# Autodesk Inventor assembly: Assembly Final
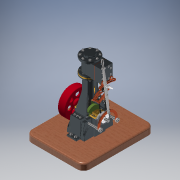
[picture p0: Inventor's stored thumbnail of the model, 180x180]
Saved by Autodesk Inventor 2017 (Build 210142000, 142)
## iProperties
Created: 2018-11-19
Part Number: Assembly Final
Document SubType Name: Assembly
Designer: Arman Grewal
Author: Arman Grewal
## Documents named in this file (56)
- C:\Users\Arman Grewal\Desktop\Engine\Assembly Final.iam
- C:\Users\Arman Grewal\Desktop\Engine\Piston.ipt
- C:\Users\Arman Grewal\Desktop\Engine\Piston Rod.ipt
- C:\Users\Arman Grewal\Documents\Inventor\Content Center Files\R2017\en-US\DIN 934\DIN 934 - M4 x 0.7.ipt
- C:\Users\Arman Grewal\Desktop\Engine\Crosshead.ipt
- C:\Users\Arman Grewal\Desktop\Engine\Crankrod.ipt
- C:\Users\Arman Grewal\Desktop\Engine\Crankrod Pin.ipt
- C:\Users\Arman Grewal\Desktop\Engine\Crankshaft outer rod.ipt
- C:\Users\Arman Grewal\Desktop\Engine\Crankshaft Center Rod.ipt
- C:\Users\Arman Grewal\Desktop\Engine\Crankshaft Counterweight.ipt
- C:\Users\Arman Grewal\Desktop\Engine\Vertical Steam Engine with Reverse Gear (anno 1830) Connecting Rod.ipt
- C:\Users\Arman Grewal\Desktop\Engine\Bearing Keeper.ipt
- C:\Users\Arman Grewal\Documents\Inventor\Content Center Files\R2017\en-US\DIN 84\DIN 84 - M3 x 8.ipt
- C:\Users\Arman Grewal\Desktop\Engine\Stand.ipt
- C:\Users\Arman Grewal\Desktop\Engine\Base cast f.ipt
- C:\Users\Arman Grewal\Documents\Inventor\Content Center Files\R2017\en-US\DIN 912\DIN 912 - M4 x 0.7 x 20 x 18.25.ipt
- C:\Users\Arman Grewal\Documents\Inventor\Content Center Files\R2017\en-US\DIN 6797  J\DIN 6797 - J 5.3.ipt
- C:\Users\Arman Grewal\Documents\Inventor\Content Center Files\R2017\en-US\DIN 934\DIN 934 - M5 x 0.8.ipt
- C:\Users\Arman Grewal\Desktop\Engine\Lower Base Bearing Holder.ipt
- C:\Users\Arman Grewal\Desktop\Engine\Upper Base Bearing Holder.ipt
- C:\Users\Arman Grewal\Documents\Inventor\Content Center Files\R2017\en-US\DIN 84\DIN 84 - M3 x 18.ipt
- C:\Users\Arman Grewal\Documents\Inventor\Content Center Files\R2017\en-US\DIN 84\DIN 84 - M3 x 20.ipt
- C:\Users\Arman Grewal\Desktop\Engine\Standard.ipt
- C:\Users\Arman Grewal\Desktop\Engine\cylinder.ipt
- C:\Users\Arman Grewal\Desktop\Engine\Upper Cylinder Cover.ipt
- C:\Users\Arman Grewal\Documents\Inventor\Content Center Files\R2017\en-US\DIN 912\DIN 912 - M3 x 0.5 x 16 x 14.75.ipt
- C:\Users\Arman Grewal\Documents\Inventor\Content Center Files\R2017\en-US\DIN 128\DIN 128 - A3.5.ipt
- C:\Users\Arman Grewal\Desktop\Engine\Lower Cylinder Cover.ipt
- C:\Users\Arman Grewal\Desktop\Engine\Upper Cylinder Packing.ipt
- C:\Users\Arman Grewal\Documents\Inventor\Content Center Files\R2017\en-US\DIN 912\DIN 912 - M3 x 0.5 x 12 x 10.75.ipt
- C:\Users\Arman Grewal\Desktop\Engine\Valve Plate.ipt
- C:\Users\Arman Grewal\Desktop\Engine\Steam Chest.ipt
- C:\Users\Arman Grewal\Desktop\Engine\Glands.ipt
- C:\Users\Arman Grewal\Desktop\Engine\Steam Chest Slide Valve Rod.ipt
- C:\Users\Arman Grewal\Desktop\Engine\Steam Chest Slide Valve.ipt
- C:\Users\Arman Grewal\Desktop\Engine\Steam Chest Cover.ipt
- C:\Users\Arman Grewal\Documents\Inventor\Content Center Files\R2017\en-US\DIN 84\DIN 84 - M2.5 x 10.ipt
- C:\Users\Arman Grewal\Documents\Inventor\Content Center Files\R2017\en-US\DIN 912\DIN 912 - M3 x 0.5 x 5 x 3.75.ipt
- C:\Users\Arman Grewal\Desktop\Engine\flywheel.ipt
- C:\Users\Arman Grewal\Desktop\Engine\Reverse Gear link 1.ipt
- C:\Users\Arman Grewal\Documents\Inventor\Content Center Files\R2017\en-US\DIN 7991(2)\DIN 7991 - M3x12.ipt
- C:\Users\Arman Grewal\Desktop\Engine\Reverse Lever.ipt
- C:\Users\Arman Grewal\Desktop\Engine\Reverse Gear Link Block.ipt
- C:\Users\Arman Grewal\Desktop\Engine\Reverse Gear Drag Link.ipt
- C:\Users\Arman Grewal\Desktop\Engine\Reverse Lever Ring Stud.ipt
- C:\Users\Arman Grewal\Desktop\Engine\Reverse Lever Ring.ipt
- C:\Users\Arman Grewal\Desktop\Engine\Reverse Gear Link Lever.ipt
- C:\Users\Arman Grewal\Desktop\Engine\Reverse Gear Link 1 updated.ipt
- C:\Users\Arman Grewal\Desktop\Engine\Reverse Gear LInk Rod.ipt
- C:\Users\Arman Grewal\Desktop\Engine\eccentric rod.ipt
- C:\Users\Arman Grewal\Desktop\Engine\eccentric.ipt
- C:\Users\Arman Grewal\Documents\Inventor\Content Center Files\R2017\en-US\DIN 84\DIN 84 - M2.5 x 8.ipt
- C:\Users\Arman Grewal\Desktop\Engine\Upper eccentric trap  lower eccentric trap (1).ipt
- C:\Users\Arman Grewal\Desktop\Engine\Upper lower eccentric trap (2).ipt
- C:\Users\Arman Grewal\Documents\Inventor\Content Center Files\R2017\en-US\AS 1427(01)\AS 1427 - M3 x 5(3).ipt
- C:\Users\Arman Grewal\Documents\Inventor\Content Center Files\R2017\en-US\DIN 934\DIN 934 - M6 x 1.ipt
## Components (140 placed, 55 different names)
1. Piston:1 — Mate:4, Insert:1, Angle:2, Mate:114, Mate:115
2. Piston Rod:1 — Mate:4, Mate:5, Mate:6, Mate:115, Mate:122
3. DIN 934 - replaced by DIN EN 24032/28673/28674 M4:1 — Insert:1
4. Crosshead:1 — Mate:5, Mate:6, Mate:7, Mate:8
5. Crankrod:1 — Mate:7, Mate:8, Mate:9, Mate:11, Mate:12
6. Crankrod Pin:1 — Mate:9
7. Crankshaft outer rod:1 — Mate:23, Mate:24, Mate:52, Mate:156, Mate:162, Rotation:2, Rotation:3
8. Crankshaft outer rod:2 — Mate:21, Mate:22, Mate:108, Flush:3
9. Crankshaft Center Rod:1 — Mate:20, Mate:25, Mate:26, Mate:27, Mate:28
10. Crankshaft Counterweight:1 — Mate:23, Mate:24, Mate:27, Mate:28, Mate:53, Rotation:1
11. Crankshaft Counterweight:2 — Mate:21, Mate:22, Mate:25, Mate:26, Mate:29
12. Vertical Steam Engine with Reverse Gear (anno 1830) Connecting Rod:1 — Mate:14, Mate:15, Mate:16, Mate:17, Mate:18, Mate:19, Mate:20, Mate:29
13. Vertical Steam Engine with Reverse Gear (anno 1830) Connecting Rod:2 — Mate:11, Mate:12, Mate:14, Mate:15, Mate:16
14. Bearing Keeper:1 — Mate:17, Mate:18, Mate:19, Insert:2, Insert:3
15. DIN 84 - replaced by DIN EN ISO 1207 M3 x 8:1 — Insert:2
16. DIN 84 - replaced by DIN EN ISO 1207 M3 x 8:2 — Insert:3
17. Stand:1 — Mate:30, Mate:31, Mate:32, Mate:33, Insert:8, Insert:9, Insert:10, Insert:11, Mate:34, Mate:36, Mate:38, Mate:40, Angle:1
18. Base cast f:1 — Mate:30, Mate:31, Mate:32, Mate:33, Insert:4, Insert:5, Insert:6, Insert:7, Mate:48, Flush:1, Mate:49, Mate:50, Flush:2, Mate:51, Mate:53, Mate:55, Mate:56, Mate:57, Mate:58, Mate:60, Mate:61, Mate:62, Mate:63, Mate:64, Mate:65, Mate:66, Mate:125, Mate:126, Mate:127, Mate:128
19. DIN 912 - replaced by DIN EN ISO 4762 M4 x 20:1 — Insert:4, Mate:42
20. DIN 912 - replaced by DIN EN ISO 4762 M4 x 20:2 — Insert:5, Mate:44
21. DIN 912 - replaced by DIN EN ISO 4762 M4 x 20:3 — Insert:6, Mate:46
22. DIN 912 - replaced by DIN EN ISO 4762 M4 x 20:4 — Insert:7
23. DIN 6797 J J 5.3:1 — Insert:8
24. DIN 6797 J J 5.3:2 — Insert:9
25. DIN 6797 J J 5.3:3 — Insert:10
26. DIN 6797 J J 5.3:4 — Insert:11, Mate:35, Mate:37, Mate:39, Mate:41
27. DIN 6797 J J 5.3:5 — Mate:34, Mate:35, Mate:43
28. DIN 6797 J J 5.3:6 — Mate:36, Mate:37, Mate:47
29. DIN 6797 J J 5.3:7 — Mate:38, Mate:39, Mate:45
30. DIN 6797 J J 5.3:8 — Mate:40, Mate:41, Insert:12, Insert:13, Insert:14, Insert:15, Insert:16, Insert:17, Insert:18, Insert:19
31. DIN 934 - replaced by DIN EN 24032/28673/28674 M5:1 — Insert:12
32. DIN 934 - replaced by DIN EN 24032/28673/28674 M5:2 — Insert:13
33. DIN 934 - replaced by DIN EN 24032/28673/28674 M5:3 — Insert:14
34. DIN 934 - replaced by DIN EN 24032/28673/28674 M5:4 — Insert:15
35. DIN 934 - replaced by DIN EN 24032/28673/28674 M5:5 — Insert:16
36. DIN 934 - replaced by DIN EN 24032/28673/28674 M5:6 — Insert:17
37. DIN 934 - replaced by DIN EN 24032/28673/28674 M5:7 — Insert:18
38. DIN 934 - replaced by DIN EN 24032/28673/28674 M5:8 — Insert:19
39. DIN 934 - replaced by DIN EN 24032/28673/28674 M4:2 — Mate:42, Mate:43
40. DIN 934 - replaced by DIN EN 24032/28673/28674 M4:3 — Mate:44, Mate:45
41. DIN 934 - replaced by DIN EN 24032/28673/28674 M4:4 — Mate:46, Mate:47
42. Lower Base Bearing Holder:1 — Mate:50, Flush:2, Mate:51, Mate:52, Mate:54
43. Lower Base Bearing Holder:2 — Mate:48, Flush:1, Mate:49, Mate:59
44. Upper Base Bearing Holder:1 — Mate:59, Mate:60, Mate:61, Mate:62, Mate:63, Insert:24, Insert:25, Insert:26, Insert:27
45. Upper Base Bearing Holder:2 — Mate:54, Mate:55, Mate:56, Mate:57, Mate:58, Insert:28, Insert:29, Insert:30, Insert:31
46. DIN 84 - replaced by DIN EN ISO 1207 M3 x 18:1 — Insert:24
47. DIN 84 - replaced by DIN EN ISO 1207 M3 x 18:2 — Insert:25
48. DIN 84 - replaced by DIN EN ISO 1207 M3 x 18:3 — Insert:26
49. DIN 84 - replaced by DIN EN ISO 1207 M3 x 18:4 — Insert:27
50. DIN 84 - replaced by DIN EN ISO 1207 M3 x 20:1 — Insert:28
51. DIN 84 - replaced by DIN EN ISO 1207 M3 x 20:2 — Insert:29
52. DIN 84 - replaced by DIN EN ISO 1207 M3 x 20:3 — Insert:30
53. DIN 84 - replaced by DIN EN ISO 1207 M3 x 20:4 — Insert:31
54. Standard:1 — Mate:64, Mate:65, Mate:66, Insert:32, Insert:33, Insert:34, Insert:35, Insert:36, Insert:37, Insert:38, Insert:39, Insert:40, Insert:41, Insert:42, Insert:43, Insert:44, Insert:45, Mate:67, Mate:68, Mate:69, Mate:70, Mate:71
55. DIN 912 - replaced by DIN EN ISO 4762 M3 x 16:1 — Insert:32
56. DIN 912 - replaced by DIN EN ISO 4762 M3 x 16:2 — Insert:33
57. DIN 912 - replaced by DIN EN ISO 4762 M3 x 16:3 — Insert:34
58. DIN 912 - replaced by DIN EN ISO 4762 M3 x 16:4 — Insert:35
59. DIN 912 - replaced by DIN EN ISO 4762 M3 x 16:5 — Insert:36
60. DIN 912 - replaced by DIN EN ISO 4762 M3 x 16:6 — Insert:37
61. DIN 128 A3.5:1 — Insert:38, Insert:50
62. DIN 128 A3.5:2 — Insert:39, Insert:49
63. DIN 128 A3.5:3 — Insert:40, Insert:51
64. DIN 128 A3.5:4 — Insert:41, Insert:46
65. DIN 128 A3.5:5 — Insert:42, Insert:47
66. DIN 128 A3.5:6 — Insert:43, Insert:52
67. DIN 128 A3.5:7 — Insert:44, Mate:85, Mate:86
68. DIN 128 A3.5:8 — Insert:45, Insert:48
69. Lower Cylinder Cover:1 — Mate:67, Mate:68, Mate:69, Mate:70, Mate:71, Mate:72, Mate:73, Mate:74, Mate:75, Mate:76, Mate:77, Mate:122
70. cylinder:1 — Mate:72, Angle:1, Mate:73, Mate:74, Mate:75, Mate:76, Mate:77, Angle:2, Mate:78, Mate:79, Mate:80, Mate:82, Mate:83, Mate:84, Mate:87, Mate:88, Mate:89, Mate:91, Mate:92, Mate:114
71. Upper Cylinder Packing:1 — Mate:78, Mate:79, Mate:80, Mate:81
72. Upper Cylinder Cover:1 — Mate:81, Mate:82, Mate:83, Mate:84, Insert:53, Insert:54, Insert:55, Insert:56, Insert:57, Insert:58, Insert:59, Insert:60, Insert:66
73. DIN 912 - replaced by DIN EN ISO 4762 M3 x 12:1 — Insert:46
74. DIN 912 - replaced by DIN EN ISO 4762 M3 x 12:2 — Mate:85, Mate:86
75. DIN 912 - replaced by DIN EN ISO 4762 M3 x 12:3 — Insert:47
76. DIN 912 - replaced by DIN EN ISO 4762 M3 x 12:4 — Insert:48
77. DIN 912 - replaced by DIN EN ISO 4762 M3 x 12:5 — Insert:49
78. DIN 912 - replaced by DIN EN ISO 4762 M3 x 12:6 — Insert:50
79. DIN 912 - replaced by DIN EN ISO 4762 M3 x 12:7 — Insert:51
80. DIN 912 - replaced by DIN EN ISO 4762 M3 x 12:8 — Insert:52
81. Valve Plate:1 — Mate:87, Mate:88, Mate:89, Mate:90, Mate:98
82. Steam Chest:1 — Mate:90, Mate:91, Mate:92, Mate:93, Mate:94, Mate:95, Angle:3, Angle:4, Mate:104, Mate:105, Mate:107, Mate:116
83. Glands:1 — Mate:93, Mate:94, Mate:95, Mate:99, Insert:69, Insert:70
84. DIN 128 A3.5:9 — Insert:53, Insert:61
85. DIN 128 A3.5:10 — Insert:54, Insert:63
86. DIN 128 A3.5:11 — Insert:55, Insert:62
87. DIN 128 A3.5:12 — Insert:56, Insert:64
88. DIN 128 A3.5:13 — Insert:57, Insert:68
89. DIN 128 A3.5:14 — Insert:58
90. DIN 128 A3.5:15 — Insert:59, Insert:67
91. DIN 128 A3.5:16 — Insert:60, Insert:65
92. DIN 912 - replaced by DIN EN ISO 4762 M3 x 12:9 — Insert:61
93. DIN 912 - replaced by DIN EN ISO 4762 M3 x 12:10 — Insert:62
94. DIN 912 - replaced by DIN EN ISO 4762 M3 x 12:11 — Insert:63
95. DIN 912 - replaced by DIN EN ISO 4762 M3 x 12:12 — Insert:64
96. DIN 912 - replaced by DIN EN ISO 4762 M3 x 12:13 — Insert:65
97. DIN 912 - replaced by DIN EN ISO 4762 M3 x 12:14 — Insert:66
98. DIN 912 - replaced by DIN EN ISO 4762 M3 x 12:15 — Insert:67
99. DIN 912 - replaced by DIN EN ISO 4762 M3 x 12:16 — Insert:68
100. Steam Chest Slide Valve Rod:1 — Mate:96, Mate:97, Angle:4, Mate:99, Mate:100, Mate:102, Mate:139, Mate:140
101. Steam Chest Slide Valve:1 — Mate:96, Mate:97, Mate:98, Angle:3, Mate:101, Mate:103, Mate:116
102. DIN 934 - replaced by DIN EN 24032/28673/28674 M4:5 — Mate:100, Mate:101
103. DIN 934 - replaced by DIN EN 24032/28673/28674 M4:6 — Mate:102, Mate:103
104. Steam Chest Cover:1 — Mate:104, Mate:105, Mate:107, Insert:71, Insert:72, Insert:73, Insert:74, Insert:75, Insert:76, Insert:77, Insert:78, Mate:117, Mate:118, Mate:119
105. DIN 84 - replaced by DIN EN ISO 1207 M2.5 x 10:1 — Insert:69
106. DIN 84 - replaced by DIN EN ISO 1207 M2.5 x 10:2 — Insert:70
107. DIN 912 - replaced by DIN EN ISO 4762 M3 x 5:1 — Insert:71
108. DIN 912 - replaced by DIN EN ISO 4762 M3 x 5:2 — Insert:72
109. DIN 912 - replaced by DIN EN ISO 4762 M3 x 5:3 — Insert:73
110. DIN 912 - replaced by DIN EN ISO 4762 M3 x 5:4 — Insert:74
111. DIN 912 - replaced by DIN EN ISO 4762 M3 x 5:5 — Insert:75
112. DIN 912 - replaced by DIN EN ISO 4762 M3 x 5:6 — Insert:76
113. DIN 912 - replaced by DIN EN ISO 4762 M3 x 5:7 — Insert:77
114. DIN 912 - replaced by DIN EN ISO 4762 M3 x 5:8 — Insert:78
115. flywheel:1 — Mate:108, Flush:3, Rotation:1
116. Reverse Lever:1 — Mate:123, Mate:124, Mate:132, Mate:133, Mate:134, Mate:146, Insert:81
117. Reverse Gear link 1:1 — Mate:117, Mate:118, Mate:119, Mate:120, Mate:121
118. DIN 7991 M3x12:1 — Mate:120
119. DIN 7991 M3x12:2 — Mate:121
120. Reverse Gear Drag Link:1 — Mate:123, Mate:124, Mate:163, Mate:164, Mate:165
121. Reverse Lever Ring Stud:1 — Mate:127, Mate:128, Mate:130, Mate:168
122. Reverse Lever Ring Stud:2 — Mate:125, Mate:126, Mate:129, Mate:166
123. Reverse Lever Ring:1 — Mate:129, Mate:130, Mate:132, Mate:146, Mate:167, Mate:169
124. Reverse Gear Link Lever:1 — Mate:133, Mate:134
125. Reverse Gear Link 1 updated:1 — Mate:138, Flush:4, Mate:141, Mate:143, Mate:147, Mate:148, Mate:149, Mate:150
126. Reverse Gear Link Block:1 — Mate:138, Flush:4, Mate:139, Mate:140
127. Reverse Gear LInk Rod:1 — Mate:141, Mate:143, Mate:163, Mate:164, Mate:165
128. eccentric rod:1 — Mate:147, Mate:148, Insert:79, Mate:154, Mate:155
129. eccentric rod:2 — Mate:149, Mate:150, Insert:80, Mate:160, Mate:161
130. DIN 84 - replaced by DIN EN ISO 1207 M2.5 x 8:1 — Insert:79
131. DIN 84 - replaced by DIN EN ISO 1207 M2.5 x 8:2 — Insert:80
132. Upper lower eccentric trap (2):3 — Mate:152, Mate:153, Flush:5
133. Upper eccentric trap  lower eccentric trap (1):1 — Mate:151, Mate:153, Flush:6, Mate:154, Mate:155
134. eccentric:1 — Mate:151, Mate:152, Flush:5, Flush:6, Mate:156, Rotation:3
135. eccentric:2 — Mate:157, Mate:158, Flush:7, Flush:8, Mate:162, Rotation:2
136. Upper lower eccentric trap (2):4 — Mate:158, Mate:159, Flush:8
137. Upper eccentric trap  lower eccentric trap (1):2 — Mate:157, Mate:159, Flush:7, Mate:160, Mate:161
138. AS 1427 - Metric M3 x 5:1 — Insert:81
139. DIN 934 - replaced by DIN EN 24032/28673/28674 M6:1 — Mate:166, Mate:167
140. DIN 934 - replaced by DIN EN 24032/28673/28674 M6:2 — Mate:168, Mate:169
## Relationships (243: Mate 151, Insert 77, Flush 8, Angle 4, RelateRotation 3)
- Mate:4: Piston:1 ↔ Piston Rod:1
- Insert:1: Piston:1 ↔ DIN 934 - replaced by DIN EN 24032/28673/28674 M4:1
- Mate:5: Piston Rod:1 ↔ Crosshead:1
- Mate:6 (-7.628 mm): Piston Rod:1 ↔ Crosshead:1
- Mate:7: Crosshead:1 ↔ Crankrod:1
- Mate:8: Crosshead:1 ↔ Crankrod:1
- Mate:9: Crankrod:1 ↔ Crankrod Pin:1
- Mate:11: Crankrod:1 ↔ Vertical Steam Engine with Reverse Gear (anno 1830) Connecting Rod:2
- Mate:12: Crankrod:1 ↔ Vertical Steam Engine with Reverse Gear (anno 1830) Connecting Rod:2
- Mate:14: Vertical Steam Engine with Reverse Gear (anno 1830) Connecting Rod:1 ↔ Vertical Steam Engine with Reverse Gear (anno 1830) Connecting Rod:2
- Mate:15: Vertical Steam Engine with Reverse Gear (anno 1830) Connecting Rod:1 ↔ Vertical Steam Engine with Reverse Gear (anno 1830) Connecting Rod:2
- Mate:16: Vertical Steam Engine with Reverse Gear (anno 1830) Connecting Rod:1 ↔ Vertical Steam Engine with Reverse Gear (anno 1830) Connecting Rod:2
- Mate:17: Vertical Steam Engine with Reverse Gear (anno 1830) Connecting Rod:1 ↔ Bearing Keeper:1
- Mate:18: Vertical Steam Engine with Reverse Gear (anno 1830) Connecting Rod:1 ↔ Bearing Keeper:1
- Mate:19: Vertical Steam Engine with Reverse Gear (anno 1830) Connecting Rod:1 ↔ Bearing Keeper:1
- Mate:20: Crankshaft Center Rod:1 ↔ Vertical Steam Engine with Reverse Gear (anno 1830) Connecting Rod:1
- Mate:21: Crankshaft outer rod:2 ↔ Crankshaft Counterweight:2
- Mate:22: Crankshaft outer rod:2 ↔ Crankshaft Counterweight:2
- Mate:23: Crankshaft outer rod:1 ↔ Crankshaft Counterweight:1
- Mate:24: Crankshaft outer rod:1 ↔ Crankshaft Counterweight:1
- Mate:25: Crankshaft Center Rod:1 ↔ Crankshaft Counterweight:2
- Mate:26: Crankshaft Center Rod:1 ↔ Crankshaft Counterweight:2
- Mate:27: Crankshaft Center Rod:1 ↔ Crankshaft Counterweight:1
- Mate:28: Crankshaft Center Rod:1 ↔ Crankshaft Counterweight:1
- Mate:29 (0.5 mm): Crankshaft Counterweight:2 ↔ Vertical Steam Engine with Reverse Gear (anno 1830) Connecting Rod:1
- Insert:2: Bearing Keeper:1 ↔ DIN 84 - replaced by DIN EN ISO 1207 M3 x 8:1
- Insert:3: Bearing Keeper:1 ↔ DIN 84 - replaced by DIN EN ISO 1207 M3 x 8:2
- Mate:30: Stand:1 ↔ Base cast f:1
- Mate:31: Stand:1 ↔ Base cast f:1
- Mate:32: Stand:1 ↔ Base cast f:1
- Mate:33: Stand:1 ↔ Base cast f:1
- Insert:4: Base cast f:1 ↔ DIN 912 - replaced by DIN EN ISO 4762 M4 x 20:1
- Insert:5: Base cast f:1 ↔ DIN 912 - replaced by DIN EN ISO 4762 M4 x 20:2
- Insert:6: Base cast f:1 ↔ DIN 912 - replaced by DIN EN ISO 4762 M4 x 20:3
- Insert:7: Base cast f:1 ↔ DIN 912 - replaced by DIN EN ISO 4762 M4 x 20:4
- Insert:8: Stand:1 ↔ DIN 6797 J J 5.3:1
- Insert:9: Stand:1 ↔ DIN 6797 J J 5.3:2
- Insert:10: Stand:1 ↔ DIN 6797 J J 5.3:3
- Insert:11: Stand:1 ↔ DIN 6797 J J 5.3:4
- Mate:34: Stand:1 ↔ DIN 6797 J J 5.3:5
- Mate:35: DIN 6797 J J 5.3:4 ↔ DIN 6797 J J 5.3:5
- Mate:36: Stand:1 ↔ DIN 6797 J J 5.3:6
- Mate:37: DIN 6797 J J 5.3:4 ↔ DIN 6797 J J 5.3:6
- Mate:38: Stand:1 ↔ DIN 6797 J J 5.3:7
- Mate:39: DIN 6797 J J 5.3:4 ↔ DIN 6797 J J 5.3:7
- Mate:40: Stand:1 ↔ DIN 6797 J J 5.3:8
- Mate:41: DIN 6797 J J 5.3:4 ↔ DIN 6797 J J 5.3:8
- Insert:12: DIN 6797 J J 5.3:8 ↔ DIN 934 - replaced by DIN EN 24032/28673/28674 M5:1
- Insert:13: DIN 6797 J J 5.3:8 ↔ DIN 934 - replaced by DIN EN 24032/28673/28674 M5:2
- Insert:14: DIN 6797 J J 5.3:8 ↔ DIN 934 - replaced by DIN EN 24032/28673/28674 M5:3
- Insert:15: DIN 6797 J J 5.3:8 ↔ DIN 934 - replaced by DIN EN 24032/28673/28674 M5:4
- Insert:16: DIN 6797 J J 5.3:8 ↔ DIN 934 - replaced by DIN EN 24032/28673/28674 M5:5
- Insert:17: DIN 6797 J J 5.3:8 ↔ DIN 934 - replaced by DIN EN 24032/28673/28674 M5:6
- Insert:18: DIN 6797 J J 5.3:8 ↔ DIN 934 - replaced by DIN EN 24032/28673/28674 M5:7
- Insert:19: DIN 6797 J J 5.3:8 ↔ DIN 934 - replaced by DIN EN 24032/28673/28674 M5:8
- Mate:42: DIN 912 - replaced by DIN EN ISO 4762 M4 x 20:1 ↔ DIN 934 - replaced by DIN EN 24032/28673/28674 M4:2
- Mate:43: DIN 6797 J J 5.3:5 ↔ DIN 934 - replaced by DIN EN 24032/28673/28674 M4:2
- Mate:44: DIN 912 - replaced by DIN EN ISO 4762 M4 x 20:2 ↔ DIN 934 - replaced by DIN EN 24032/28673/28674 M4:3
- Mate:45: DIN 6797 J J 5.3:7 ↔ DIN 934 - replaced by DIN EN 24032/28673/28674 M4:3
- Mate:46: DIN 912 - replaced by DIN EN ISO 4762 M4 x 20:3 ↔ DIN 934 - replaced by DIN EN 24032/28673/28674 M4:4
- Mate:47: DIN 6797 J J 5.3:6 ↔ DIN 934 - replaced by DIN EN 24032/28673/28674 M4:4
- Mate:48: Base cast f:1 ↔ Lower Base Bearing Holder:2
- Flush:1: Base cast f:1 ↔ Lower Base Bearing Holder:2
- Mate:49: Base cast f:1 ↔ Lower Base Bearing Holder:2
- Mate:50: Base cast f:1 ↔ Lower Base Bearing Holder:1
- Flush:2: Base cast f:1 ↔ Lower Base Bearing Holder:1
- Mate:51: Base cast f:1 ↔ Lower Base Bearing Holder:1
- Mate:52: Crankshaft outer rod:1 ↔ Lower Base Bearing Holder:1
- Mate:53 (2.5 mm): Crankshaft Counterweight:1 ↔ Base cast f:1
- Mate:54: Lower Base Bearing Holder:1 ↔ Upper Base Bearing Holder:2
- Mate:55: Base cast f:1 ↔ Upper Base Bearing Holder:2
- Mate:56: Base cast f:1 ↔ Upper Base Bearing Holder:2
- Mate:57: Base cast f:1 ↔ Upper Base Bearing Holder:2
- Mate:58: Base cast f:1 ↔ Upper Base Bearing Holder:2
- Mate:59: Lower Base Bearing Holder:2 ↔ Upper Base Bearing Holder:1
- Mate:60: Base cast f:1 ↔ Upper Base Bearing Holder:1
- Mate:61: Base cast f:1 ↔ Upper Base Bearing Holder:1
- Mate:62: Base cast f:1 ↔ Upper Base Bearing Holder:1
- Mate:63: Base cast f:1 ↔ Upper Base Bearing Holder:1
- Insert:24: Upper Base Bearing Holder:1 ↔ DIN 84 - replaced by DIN EN ISO 1207 M3 x 18:1
- Insert:25: Upper Base Bearing Holder:1 ↔ DIN 84 - replaced by DIN EN ISO 1207 M3 x 18:2
- Insert:26: Upper Base Bearing Holder:1 ↔ DIN 84 - replaced by DIN EN ISO 1207 M3 x 18:3
- Insert:27: Upper Base Bearing Holder:1 ↔ DIN 84 - replaced by DIN EN ISO 1207 M3 x 18:4
- Insert:28: Upper Base Bearing Holder:2 ↔ DIN 84 - replaced by DIN EN ISO 1207 M3 x 20:1
- Insert:29: Upper Base Bearing Holder:2 ↔ DIN 84 - replaced by DIN EN ISO 1207 M3 x 20:2
- Insert:30: Upper Base Bearing Holder:2 ↔ DIN 84 - replaced by DIN EN ISO 1207 M3 x 20:3
- Insert:31: Upper Base Bearing Holder:2 ↔ DIN 84 - replaced by DIN EN ISO 1207 M3 x 20:4
- Mate:64: Base cast f:1 ↔ Standard:1
- Mate:65: Base cast f:1 ↔ Standard:1
- Mate:66: Base cast f:1 ↔ Standard:1
- Insert:32: Standard:1 ↔ DIN 912 - replaced by DIN EN ISO 4762 M3 x 16:1
- Insert:33: Standard:1 ↔ DIN 912 - replaced by DIN EN ISO 4762 M3 x 16:2
- Insert:34: Standard:1 ↔ DIN 912 - replaced by DIN EN ISO 4762 M3 x 16:3
- Insert:35: Standard:1 ↔ DIN 912 - replaced by DIN EN ISO 4762 M3 x 16:4
- Insert:36: Standard:1 ↔ DIN 912 - replaced by DIN EN ISO 4762 M3 x 16:5
- Insert:37: Standard:1 ↔ DIN 912 - replaced by DIN EN ISO 4762 M3 x 16:6
- Insert:38: Standard:1 ↔ DIN 128 A3.5:1
- Insert:39: Standard:1 ↔ DIN 128 A3.5:2
- Insert:40: Standard:1 ↔ DIN 128 A3.5:3
- Insert:41: Standard:1 ↔ DIN 128 A3.5:4
- Insert:42: Standard:1 ↔ DIN 128 A3.5:5
- Insert:43: Standard:1 ↔ DIN 128 A3.5:6
- Insert:44: Standard:1 ↔ DIN 128 A3.5:7
- Insert:45: Standard:1 ↔ DIN 128 A3.5:8
- Mate:67: Standard:1 ↔ Lower Cylinder Cover:1
- Mate:68: Standard:1 ↔ Lower Cylinder Cover:1
- Mate:69: Standard:1 ↔ Lower Cylinder Cover:1
- Mate:70: Standard:1 ↔ Lower Cylinder Cover:1
- Mate:71: Standard:1 ↔ Lower Cylinder Cover:1
- Mate:72: Lower Cylinder Cover:1 ↔ cylinder:1
- Angle:1 (0 deg): Stand:1 ↔ cylinder:1
- Mate:73: Lower Cylinder Cover:1 ↔ cylinder:1
- Mate:74: Lower Cylinder Cover:1 ↔ cylinder:1
- Mate:75: Lower Cylinder Cover:1 ↔ cylinder:1
- Mate:76: Lower Cylinder Cover:1 ↔ cylinder:1
- Mate:77: Lower Cylinder Cover:1 ↔ cylinder:1
- Angle:2 (0 deg): Piston:1 ↔ cylinder:1
- Mate:78: cylinder:1 ↔ Upper Cylinder Packing:1
- Mate:79: cylinder:1 ↔ Upper Cylinder Packing:1
- Mate:80: cylinder:1 ↔ Upper Cylinder Packing:1
- Mate:81: Upper Cylinder Packing:1 ↔ Upper Cylinder Cover:1
- Mate:82: cylinder:1 ↔ Upper Cylinder Cover:1
- Mate:83: cylinder:1 ↔ Upper Cylinder Cover:1
- Mate:84: cylinder:1 ↔ Upper Cylinder Cover:1
- Insert:46: DIN 128 A3.5:4 ↔ DIN 912 - replaced by DIN EN ISO 4762 M3 x 12:1
- Mate:85: DIN 128 A3.5:7 ↔ DIN 912 - replaced by DIN EN ISO 4762 M3 x 12:2
- Mate:86: DIN 128 A3.5:7 ↔ DIN 912 - replaced by DIN EN ISO 4762 M3 x 12:2
- Insert:47: DIN 128 A3.5:5 ↔ DIN 912 - replaced by DIN EN ISO 4762 M3 x 12:3
- Insert:48: DIN 128 A3.5:8 ↔ DIN 912 - replaced by DIN EN ISO 4762 M3 x 12:4
- Insert:49: DIN 128 A3.5:2 ↔ DIN 912 - replaced by DIN EN ISO 4762 M3 x 12:5
- Insert:50: DIN 128 A3.5:1 ↔ DIN 912 - replaced by DIN EN ISO 4762 M3 x 12:6
- Insert:51: DIN 128 A3.5:3 ↔ DIN 912 - replaced by DIN EN ISO 4762 M3 x 12:7
- Insert:52: DIN 128 A3.5:6 ↔ DIN 912 - replaced by DIN EN ISO 4762 M3 x 12:8
- Mate:87: cylinder:1 ↔ Valve Plate:1
- Mate:88: cylinder:1 ↔ Valve Plate:1
- Mate:89: cylinder:1 ↔ Valve Plate:1
- Mate:90: Valve Plate:1 ↔ Steam Chest:1
- Mate:91: cylinder:1 ↔ Steam Chest:1
- Mate:92: cylinder:1 ↔ Steam Chest:1
- Mate:93: Steam Chest:1 ↔ Glands:1
- Mate:94: Steam Chest:1 ↔ Glands:1
- Mate:95: Steam Chest:1 ↔ Glands:1
- Insert:53: Upper Cylinder Cover:1 ↔ DIN 128 A3.5:9
- Insert:54: Upper Cylinder Cover:1 ↔ DIN 128 A3.5:10
- Insert:55: Upper Cylinder Cover:1 ↔ DIN 128 A3.5:11
- Insert:56: Upper Cylinder Cover:1 ↔ DIN 128 A3.5:12
- Insert:57: Upper Cylinder Cover:1 ↔ DIN 128 A3.5:13
- Insert:58: Upper Cylinder Cover:1 ↔ DIN 128 A3.5:14
- Insert:59: Upper Cylinder Cover:1 ↔ DIN 128 A3.5:15
- Insert:60: Upper Cylinder Cover:1 ↔ DIN 128 A3.5:16
- Insert:61: DIN 128 A3.5:9 ↔ DIN 912 - replaced by DIN EN ISO 4762 M3 x 12:9
- Insert:62: DIN 128 A3.5:11 ↔ DIN 912 - replaced by DIN EN ISO 4762 M3 x 12:10
- Insert:63: DIN 128 A3.5:10 ↔ DIN 912 - replaced by DIN EN ISO 4762 M3 x 12:11
- Insert:64: DIN 128 A3.5:12 ↔ DIN 912 - replaced by DIN EN ISO 4762 M3 x 12:12
- Insert:65: DIN 128 A3.5:16 ↔ DIN 912 - replaced by DIN EN ISO 4762 M3 x 12:13
- Insert:66: Upper Cylinder Cover:1 ↔ DIN 912 - replaced by DIN EN ISO 4762 M3 x 12:14
- Insert:67: DIN 128 A3.5:15 ↔ DIN 912 - replaced by DIN EN ISO 4762 M3 x 12:15
- Insert:68: DIN 128 A3.5:13 ↔ DIN 912 - replaced by DIN EN ISO 4762 M3 x 12:16
- Mate:96: Steam Chest Slide Valve Rod:1 ↔ Steam Chest Slide Valve:1
- Mate:97 (2.844 mm): Steam Chest Slide Valve Rod:1 ↔ Steam Chest Slide Valve:1
- Mate:98: Valve Plate:1 ↔ Steam Chest Slide Valve:1
- Angle:3 (0 deg): Steam Chest:1 ↔ Steam Chest Slide Valve:1
- Angle:4 (0 deg): Steam Chest:1 ↔ Steam Chest Slide Valve Rod:1
- Mate:99: Glands:1 ↔ Steam Chest Slide Valve Rod:1
- Mate:100: Steam Chest Slide Valve Rod:1 ↔ DIN 934 - replaced by DIN EN 24032/28673/28674 M4:5
- Mate:101: Steam Chest Slide Valve:1 ↔ DIN 934 - replaced by DIN EN 24032/28673/28674 M4:5
- Mate:102: Steam Chest Slide Valve Rod:1 ↔ DIN 934 - replaced by DIN EN 24032/28673/28674 M4:6
- Mate:103: Steam Chest Slide Valve:1 ↔ DIN 934 - replaced by DIN EN 24032/28673/28674 M4:6
- Mate:104: Steam Chest:1 ↔ Steam Chest Cover:1
- Mate:105: Steam Chest:1 ↔ Steam Chest Cover:1
- Mate:107: Steam Chest:1 ↔ Steam Chest Cover:1
- Insert:69: Glands:1 ↔ DIN 84 - replaced by DIN EN ISO 1207 M2.5 x 10:1
- Insert:70: Glands:1 ↔ DIN 84 - replaced by DIN EN ISO 1207 M2.5 x 10:2
- Insert:71: Steam Chest Cover:1 ↔ DIN 912 - replaced by DIN EN ISO 4762 M3 x 5:1
- Insert:72: Steam Chest Cover:1 ↔ DIN 912 - replaced by DIN EN ISO 4762 M3 x 5:2
- Insert:73: Steam Chest Cover:1 ↔ DIN 912 - replaced by DIN EN ISO 4762 M3 x 5:3
- Insert:74: Steam Chest Cover:1 ↔ DIN 912 - replaced by DIN EN ISO 4762 M3 x 5:4
- Insert:75: Steam Chest Cover:1 ↔ DIN 912 - replaced by DIN EN ISO 4762 M3 x 5:5
- Insert:76: Steam Chest Cover:1 ↔ DIN 912 - replaced by DIN EN ISO 4762 M3 x 5:6
- Insert:77: Steam Chest Cover:1 ↔ DIN 912 - replaced by DIN EN ISO 4762 M3 x 5:7
- Insert:78: Steam Chest Cover:1 ↔ DIN 912 - replaced by DIN EN ISO 4762 M3 x 5:8
- Mate:108: Crankshaft outer rod:2 ↔ flywheel:1
- Flush:3: Crankshaft outer rod:2 ↔ flywheel:1
- Mate:114: Piston:1 ↔ cylinder:1
- Mate:115: Piston:1 ↔ Piston Rod:1
- Mate:116: Steam Chest:1 ↔ Steam Chest Slide Valve:1
- Mate:117: Steam Chest Cover:1 ↔ Reverse Gear link 1:1
- Mate:118: Steam Chest Cover:1 ↔ Reverse Gear link 1:1
- Mate:119: Steam Chest Cover:1 ↔ Reverse Gear link 1:1
- Mate:120: Reverse Gear link 1:1 ↔ DIN 7991 M3x12:1
- Mate:121: Reverse Gear link 1:1 ↔ DIN 7991 M3x12:2
- Mate:122: Piston Rod:1 ↔ Lower Cylinder Cover:1
- Mate:123: Reverse Lever:1 ↔ Reverse Gear Drag Link:1
- Mate:124: Reverse Lever:1 ↔ Reverse Gear Drag Link:1
- Mate:125: Base cast f:1 ↔ Reverse Lever Ring Stud:2
- Mate:126: Base cast f:1 ↔ Reverse Lever Ring Stud:2
- Mate:127: Base cast f:1 ↔ Reverse Lever Ring Stud:1
- Mate:128: Base cast f:1 ↔ Reverse Lever Ring Stud:1
- Mate:129: Reverse Lever Ring Stud:2 ↔ Reverse Lever Ring:1
- Mate:130: Reverse Lever Ring Stud:1 ↔ Reverse Lever Ring:1
- Mate:132: Reverse Lever:1 ↔ Reverse Lever Ring:1
- Mate:133: Reverse Lever:1 ↔ Reverse Gear Link Lever:1
- Mate:134: Reverse Lever:1 ↔ Reverse Gear Link Lever:1
- Rotation:1 [RelateRotation] (1 ul): Crankshaft Counterweight:1 ↔ flywheel:1
- Mate:138: Reverse Gear Link 1 updated:1 ↔ Reverse Gear Link Block:1
- Flush:4: Reverse Gear Link 1 updated:1 ↔ Reverse Gear Link Block:1
- Mate:139: Steam Chest Slide Valve Rod:1 ↔ Reverse Gear Link Block:1
- Mate:140: Steam Chest Slide Valve Rod:1 ↔ Reverse Gear Link Block:1
- Mate:141: Reverse Gear Link 1 updated:1 ↔ Reverse Gear LInk Rod:1
- Mate:143: Reverse Gear Link 1 updated:1 ↔ Reverse Gear LInk Rod:1
- Mate:146: Reverse Lever:1 ↔ Reverse Lever Ring:1
- Mate:147: Reverse Gear Link 1 updated:1 ↔ eccentric rod:1
- Mate:148: Reverse Gear Link 1 updated:1 ↔ eccentric rod:1
- Mate:149: Reverse Gear Link 1 updated:1 ↔ eccentric rod:2
- Mate:150: Reverse Gear Link 1 updated:1 ↔ eccentric rod:2
- Insert:79: eccentric rod:1 ↔ DIN 84 - replaced by DIN EN ISO 1207 M2.5 x 8:1
- Insert:80: eccentric rod:2 ↔ DIN 84 - replaced by DIN EN ISO 1207 M2.5 x 8:2
- Mate:151: Upper eccentric trap  lower eccentric trap (1):1 ↔ eccentric:1
- Mate:152: Upper lower eccentric trap (2):3 ↔ eccentric:1
- Mate:153: Upper lower eccentric trap (2):3 ↔ Upper eccentric trap  lower eccentric trap (1):1
- Flush:5: Upper lower eccentric trap (2):3 ↔ eccentric:1
- Flush:6: Upper eccentric trap  lower eccentric trap (1):1 ↔ eccentric:1
- Mate:154: eccentric rod:1 ↔ Upper eccentric trap  lower eccentric trap (1):1
- Mate:155: eccentric rod:1 ↔ Upper eccentric trap  lower eccentric trap (1):1
- Mate:156: Crankshaft outer rod:1 ↔ eccentric:1
- Mate:157: eccentric:2 ↔ Upper eccentric trap  lower eccentric trap (1):2
- Mate:158: eccentric:2 ↔ Upper lower eccentric trap (2):4
- Mate:159: Upper lower eccentric trap (2):4 ↔ Upper eccentric trap  lower eccentric trap (1):2
- Flush:7: eccentric:2 ↔ Upper eccentric trap  lower eccentric trap (1):2
- Flush:8: eccentric:2 ↔ Upper lower eccentric trap (2):4
- Mate:160: eccentric rod:2 ↔ Upper eccentric trap  lower eccentric trap (1):2
- Mate:161: eccentric rod:2 ↔ Upper eccentric trap  lower eccentric trap (1):2
- Mate:162: Crankshaft outer rod:1 ↔ eccentric:2
- Rotation:2 [RelateRotation] (1 ul): Crankshaft outer rod:1 ↔ eccentric:2
- Rotation:3 [RelateRotation] (1 ul): Crankshaft outer rod:1 ↔ eccentric:1
- Mate:163: Reverse Gear Drag Link:1 ↔ Reverse Gear LInk Rod:1
- Mate:164: Reverse Gear Drag Link:1 ↔ Reverse Gear LInk Rod:1
- Mate:165: Reverse Gear Drag Link:1 ↔ Reverse Gear LInk Rod:1
- Insert:81: Reverse Lever:1 ↔ AS 1427 - Metric M3 x 5:1
- Mate:166: Reverse Lever Ring Stud:2 ↔ DIN 934 - replaced by DIN EN 24032/28673/28674 M6:1
- Mate:167: Reverse Lever Ring:1 ↔ DIN 934 - replaced by DIN EN 24032/28673/28674 M6:1
- Mate:168: Reverse Lever Ring Stud:1 ↔ DIN 934 - replaced by DIN EN 24032/28673/28674 M6:2
- Mate:169: Reverse Lever Ring:1 ↔ DIN 934 - replaced by DIN EN 24032/28673/28674 M6:2
